# Autodesk Inventor assembly: leg_ass_1
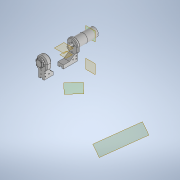
[picture p0: Inventor's stored thumbnail of the model, 180x180]
Saved by Autodesk Inventor 2020 (Build 240168000, 168)
## iProperties
Created: 2019-05-04
Part Number: leg_ass_1
Document SubType Name: Assembly
Designer: psrob
Author: psrob
## Documents named in this file (5)
- E:\projects-2\project dog gen2\hardware\leg_ass_1.iam
- E:\projects-2\project dog gen2\hardware\dog_bone_1.ipt
- E:\projects-2\project dog gen2\hardware\motor_2.ipt
- E:\projects-2\project dog gen2\hardware\dog_bone_3.ipt
- E:\projects-2\project dog gen2\hardware\encoder_ass.iam
## Components (4 placed, 4 different names)
1. dog_bone_1:1 — Flush:1, Angle:1, Insert:10, Insert:11
2. motor_2:1 — Mate:1, Tangent:1, Flush:2
3. dog_bone_3:1 — Flush:1, Mate:1, Angle:1, Tangent:1
4. encoder_ass:1 [sub-assembly] — Insert:10, Insert:11
## Relationships (7: Flush 2, Insert 2, Mate 1, Angle 1, Tangent 1)
- Flush:1: dog_bone_1:1 ↔ dog_bone_3:1
- Mate:1: motor_2:1 ↔ dog_bone_3:1
- Angle:1 (0 deg): dog_bone_1:1 ↔ dog_bone_3:1
- Tangent:1: motor_2:1 ↔ dog_bone_3:1
- Insert:10: dog_bone_1:1 ↔ encoder_ass:1
- Insert:11: dog_bone_1:1 ↔ encoder_ass:1
- Flush:2 (-10 mm): motor_2:1
